# Autodesk Inventor assembly: GX 160
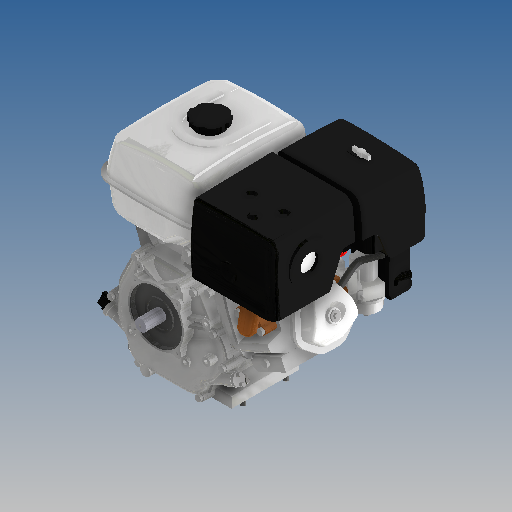
[picture p0: Inventor's stored thumbnail of the model, 512x512]
Saved by Autodesk Inventor 2021.1 (Build 251245000, 245)
## iProperties
Created: 2020-09-03
Part Number: GX 160
Document SubType Name: Assembly
Designer: alid
Description: Honda GX160 Engine
Author: alid
Revision Number: A
## Documents named in this file (3)
- C:\Vault Workspace\Design Data\Projects\PRJ0095\PWTR-Components\PWTR-Supplier\GX 160.iam
- C:\Vault Workspace\Design Data\Projects\PRJ0095\PWTR-Components\PWTR-Supplier\PWTR-0075.ipt
- C:\Vault Workspace\Design Data\Projects\PRJ0095\PWTR-Components\PWTR-Supplier\PWTR-0133.ipt
## Components (5 placed, 2 different names)
1. EngineBlock — Insert:1
2. PWTR-0133:1 — Insert:1
3. PWTR-0133:2
4. PWTR-0133:3
5. PWTR-0133:4
## Component patterns: (4 elements, first: PWTR-0133:1)
## Relationships (1: Insert 1)
- Insert:1: EngineBlock ↔ PWTR-0133:1
